# Autodesk Inventor assembly: MotorMount
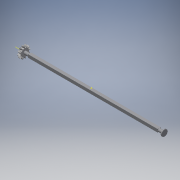
[picture p0: Inventor's stored thumbnail of the model, 180x180]
Saved by Autodesk Inventor 2017 (Build 210142000, 142)
## iProperties
Created: 2017-01-26
Part Number: MotorMount
Document SubType Name: Assembly
Designer: David Kopala
Author: David Kopala
## Documents named in this file (3)
- Z:\Documents\Drone\Drone\3D Models\Project\Chassis_04\MotorMount.iam
- Z:\Documents\Drone\Drone\3D Models\Project\Chassis_04\MotorMntPart.ipt
- Z:\Documents\Drone\Drone\3D Models\Project\Chassis_04\BevelGear_Ref\Design Accelerator\Bevel Gear23.ipt
## Components (2 placed, 2 different names)
1. MotorMntPart:1 — Insert:1
2. Bevel Gear2:1 — Insert:1
## Relationships (1: Insert 1)
- Insert:1: MotorMntPart:1 ↔ Bevel Gear2:1
